# Autodesk Inventor assembly: Assembly
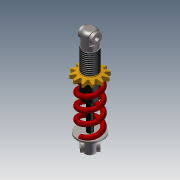
[picture p0: Inventor's stored thumbnail of the model, 180x180]
Saved by Autodesk Inventor 2015 (Build 190159000, 159)
## iProperties
Created: 2021-04-19
Part Number: Assembly
Document SubType Name: Assembly
Designer: Diptanshu Das
Title: Assembly.STEP
Description: STEP AP214
Creation Date: 2021-04-19
Sending System: SolidWorks 2020
Preprocessor: SwSTEP 2.0
Author: Diptanshu Das
## Documents named in this file (5)
- D:\SW_design\INVENTOR\Shock Absorber\Assembly\Assembly.iam
- D:\SW_design\INVENTOR\Shock Absorber\Assembly\top rod.ipt
- D:\SW_design\INVENTOR\Shock Absorber\Assembly\base.ipt
- D:\SW_design\INVENTOR\Shock Absorber\Assembly\nut.ipt
- D:\SW_design\INVENTOR\Shock Absorber\Assembly\spring.ipt
## Components (4 placed, 4 different names)
1. top rod_1 — Mate:1, Flush:1, Mate:2, Mate:6, Mate:9, Mate:10
2. base_2 — Mate:2, Mate:6, Mate:7
3. nut_3 — Mate:1, Flush:1, Mate:5
4. spring:1 — Mate:5, Mate:7, Mate:9, Mate:10
## Relationships (8: Mate 7, Flush 1)
- Mate:1: top rod_1 ↔ nut_3
- Flush:1 (35 mm): top rod_1 ↔ nut_3
- Mate:2: top rod_1 ↔ base_2
- Mate:5: nut_3 ↔ spring:1
- Mate:6 (49 mm): top rod_1 ↔ base_2
- Mate:7: base_2 ↔ spring:1
- Mate:9: top rod_1 ↔ spring:1
- Mate:10: top rod_1 ↔ spring:1
